# Autodesk Inventor assembly: Сборка штурвал
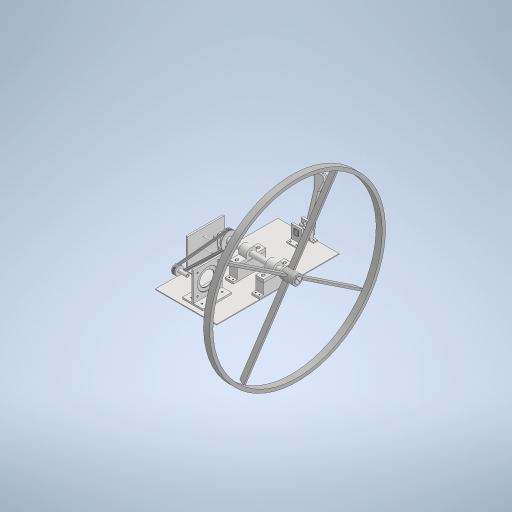
[picture p0: Inventor's stored thumbnail of the model, 512x512]
Saved by Autodesk Inventor 2023 (Build 270158000, 158)
## iProperties
Created: 2022-05-01
Part Number: Сборка штурвал
Document SubType Name: Assembly
Designer: User
Author: User
## Documents named in this file (19)
- D:\Стойка\VR-simulator-3D-models\Механизм\Сборка штурвал.iam
- D:\Стойка\VR-simulator-3D-models\Механизм\Маховик.ipt
- D:\Стойка\VR-simulator-3D-models\Механизм\Вал.ipt
- D:\Стойка\VR-simulator-3D-models\Механизм\Диск (маховик, вал).ipt
- D:\Стойка\VR-simulator-3D-models\Механизм\Стена 16 мм отверстие.ipt
- D:\Стойка\VR-simulator-3D-models\Механизм\Механизм.ipt
- D:\Стойка\VR-simulator-3D-models\Механизм\Подшипник с лапками.ipt
- D:\Стойка\VR-simulator-3D-models\Механизм ручки\Сборка ручка.iam
- D:\Стойка\VR-simulator-3D-models\Механизм\Шкив 80.ipt
- D:\Стойка\VR-simulator-3D-models\Механизм\Подставка подшипника.ipt
- D:\Стойка\VR-simulator-3D-models\Механизм\Шкив 20.ipt
- D:\Стойка\VR-simulator-3D-models\Механизм\Кронштейн мотора.ipt
- D:\Стойка\VR-simulator-3D-models\Механизм\Ограничитель.ipt
- D:\Стойка\VR-simulator-3D-models\Механизм\Стенка энкодера штурвала.ipt
- D:\Стойка\VR-simulator-3D-models\Механизм\Part38.ipt
- D:\Стойка\VR-simulator-3D-models\Механизм\Втулка энкодера штурвала.ipt
- D:\Стойка\VR-simulator-3D-models\Механизм\Штурвал.ipt
- D:\Стойка\VR-simulator-3D-models\Механизм\Болт маховика.ipt
- D:\Стойка\VR-simulator-3D-models\Механизм\Сборка штурвал\Мастер проектирования\Передача клиновым ремнем2.iam
## Components (21 placed, 18 different names)
1. Стена 16 мм отверстие:1 — Заподлицо:1
2. Стена 16 мм отверстие:2 — Заподлицо:1
3. Механизм:1 — Совмещение:18, Заподлицо:2, Совмещение:31, Совмещение:32, Заподлицо:7, Совмещение:38, Совмещение:40, Совмещение:41, Совмещение:42, Заподлицо:8, Совмещение:58
4. Подшипник с лапками:1 — Цилиндрический:22, Заподлицо:5, Заподлицо:6
5. Подшипник с лапками:2 — Цилиндрический:22, Совмещение:21, Заподлицо:3, Совмещение:33, Заподлицо:4
6. Сборка ручка:1 [sub-assembly] — Совмещение:18, Заподлицо:2, Совмещение:42
7. Вал:1 — Совмещение:21, Совмещение:22, Совмещение:23, Совмещение:24, Совмещение:28, Совмещение:43, Совмещение:46, Совмещение:48
8. Диск (маховик, вал):1 — Совмещение:22, Совмещение:23, Совмещение:24, Совмещение:25, Совмещение:26, Совмещение:27, Совмещение:30, С поворотом:2
9. Маховик:1 — Совмещение:25, Совмещение:26, Совмещение:27, Совмещение:30, Совмещение:56, Совмещение:57, С поворотом:2
10. Шкив 80:1 — Совмещение:28, Совмещение:43, Совмещение:49, Вставка:1, С поворотом:4
11. Подставка подшипника:1 — Совмещение:31, Заподлицо:5, Заподлицо:6
12. Подставка подшипника:2 — Совмещение:32, Заподлицо:3, Совмещение:33, Заподлицо:4, Заподлицо:7, Совмещение:40, Совмещение:41
13. Шкив 20:1 — С поворотом:3, С поворотом:5
14. Кронштейн мотора:1 — Совмещение:38
15. Стенка энкодера штурвала:1 — Заподлицо:8, Совмещение:45, Совмещение:47, Совмещение:58
16. Part38:1 — Совмещение:45, Совмещение:46, Совмещение:47, Совмещение:50, Совмещение:51
17. Втулка энкодера штурвала:1 — Совмещение:48, Совмещение:49, Совмещение:50, Совмещение:51, Совмещение:52, Совмещение:53, Касательность:1
18. Ограничитель:1 — Совмещение:52, Совмещение:53, Касательность:1
19. Штурвал:1 — Совмещение:54, Совмещение:55, Совмещение:56, Совмещение:57
20. Болт маховика:1 — Совмещение:54, Совмещение:55
21. Передача клиновым ремнем:1 [sub-assembly] — С поворотом:3, Вставка:1, С поворотом:4, С поворотом:5
## Relationships (47: Mate 32, Flush 8, RevoluteJoint 4, CylindricalJoint 1, Tangent 1, Insert 1)
- Заподлицо:1 [Flush]: Стена 16 мм отверстие:1 ↔ Стена 16 мм отверстие:2
- Совмещение:18 [Mate]: Механизм:1 ↔ Сборка ручка:1
- Заподлицо:2 [Flush]: Механизм:1 ↔ Сборка ручка:1
- Цилиндрический:22 [CylindricalJoint]: Подшипник с лапками:1 ↔ Подшипник с лапками:2
- Совмещение:21 [Mate]: Подшипник с лапками:2 ↔ Вал:1
- Совмещение:22 [Mate]: Вал:1 ↔ Диск (маховик, вал):1
- Совмещение:23 [Mate]: Вал:1 ↔ Диск (маховик, вал):1
- Совмещение:24 [Mate]: Вал:1 ↔ Диск (маховик, вал):1
- Совмещение:25 [Mate]: Диск (маховик, вал):1 ↔ Маховик:1
- Совмещение:26 [Mate]: Диск (маховик, вал):1 ↔ Маховик:1
- Совмещение:27 [Mate]: Диск (маховик, вал):1 ↔ Маховик:1
- Совмещение:28 [Mate]: Вал:1 ↔ Шкив 80:1
- Совмещение:30 [Mate]: Диск (маховик, вал):1 ↔ Маховик:1
- Совмещение:31 [Mate]: Механизм:1 ↔ Подставка подшипника:1
- Совмещение:32 [Mate]: Механизм:1 ↔ Подставка подшипника:2
- Заподлицо:3 [Flush]: Подшипник с лапками:2 ↔ Подставка подшипника:2
- Совмещение:33 [Mate]: Подшипник с лапками:2 ↔ Подставка подшипника:2
- Заподлицо:4 [Flush]: Подшипник с лапками:2 ↔ Подставка подшипника:2
- Заподлицо:5 [Flush]: Подшипник с лапками:1 ↔ Подставка подшипника:1
- Заподлицо:6 [Flush]: Подшипник с лапками:1 ↔ Подставка подшипника:1
- Заподлицо:7 [Flush]: Механизм:1 ↔ Подставка подшипника:2
- Совмещение:38 [Mate]: Механизм:1 ↔ Кронштейн мотора:1
- Совмещение:40 [Mate]: Механизм:1 ↔ Подставка подшипника:2
- Совмещение:41 [Mate]: Механизм:1 ↔ Подставка подшипника:2
- Совмещение:42 [Mate]: Механизм:1 ↔ Сборка ручка:1
- Совмещение:43 [Mate]: Вал:1 ↔ Шкив 80:1
- Заподлицо:8 [Flush]: Механизм:1 ↔ Стенка энкодера штурвала:1
- Совмещение:45 [Mate]: Стенка энкодера штурвала:1 ↔ Part38:1
- Совмещение:46 [Mate]: Вал:1 ↔ Part38:1
- Совмещение:47 [Mate]: Стенка энкодера штурвала:1 ↔ Part38:1
- Совмещение:48 [Mate]: Вал:1 ↔ Втулка энкодера штурвала:1
- Совмещение:49 [Mate]: Шкив 80:1 ↔ Втулка энкодера штурвала:1
- Совмещение:50 [Mate]: Part38:1 ↔ Втулка энкодера штурвала:1
- Совмещение:51 [Mate]: Part38:1 ↔ Втулка энкодера штурвала:1
- Совмещение:52 [Mate]: Втулка энкодера штурвала:1 ↔ Ограничитель:1
- Совмещение:53 [Mate]: Втулка энкодера штурвала:1 ↔ Ограничитель:1
- Касательность:1 [Tangent]: Втулка энкодера штурвала:1 ↔ Ограничитель:1
- Совмещение:54 [Mate]: Штурвал:1 ↔ Болт маховика:1
- Совмещение:55 [Mate]: Штурвал:1 ↔ Болт маховика:1
- Совмещение:56 [Mate]: Маховик:1 ↔ Штурвал:1
- Совмещение:57 [Mate]: Маховик:1 ↔ Штурвал:1
- Совмещение:58 [Mate]: Механизм:1 ↔ Стенка энкодера штурвала:1
- С поворотом:2 [RevoluteJoint]: Диск (маховик, вал):1 ↔ Маховик:1
- С поворотом:3 [RevoluteJoint]: Шкив 20:1 ↔ Передача клиновым ремнем:1
- Вставка:1 [Insert]: Шкив 80:1 ↔ Передача клиновым ремнем:1
- С поворотом:4 [RevoluteJoint]: Шкив 80:1 ↔ Передача клиновым ремнем:1
- С поворотом:5 [RevoluteJoint]: Шкив 20:1 ↔ Передача клиновым ремнем:1
